# Autodesk Inventor assembly: PCB-HousingAssembly
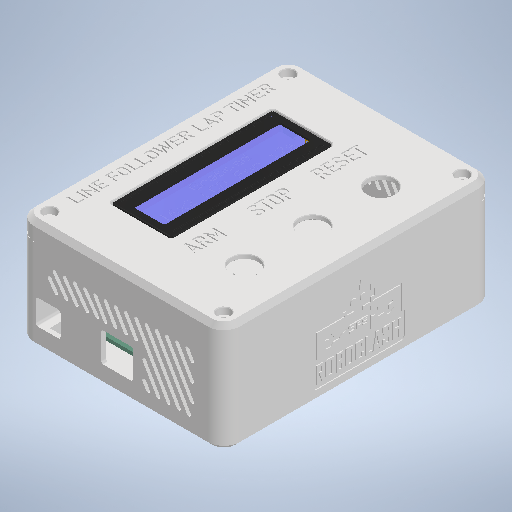
[picture p0: Inventor's stored thumbnail of the model, 512x512]
Saved by Autodesk Inventor 2025.1 (Build 291241000, 241)
## iProperties
Created: 2025-03-29
Part Number: PCB-HousingAssembly
Document SubType Name: Assembly
Designer: 42060
Author: 42060
## Documents named in this file (5)
- C:\Users\42060\Desktop\School\Projects\RoboClash\LineFolloweLapTimer_HousingBottom\PCB-HousingAssembly.iam
- C:\Users\42060\Desktop\School\Projects\RoboClash\LineFolloweLapTimer_HousingBottom\LCD.iam
- C:\Users\42060\Desktop\School\Projects\RoboClash\LineFolloweLapTimer_HousingBottom\PCB-HousingBottom.ipt
- C:\Users\42060\Desktop\School\Projects\RoboClash\LineFolloweLapTimer_HousingBottom\PCB-HousingTop.ipt
- C:\Users\42060\Desktop\School\Projects\RoboClash\LineFolloweLapTimer_HousingBottom\LF_LAP_TIMER.iam
## Components (4 placed, 4 different names)
1. LCD:1 [sub-assembly] — Vložit:2, Vložit:3
2. PCB-HousingBottom:1 — Stejný směr:1, Stejný směr:2, Proti sobě:1, Vložit:4, Úhel:1
3. PCB-HousingTop:1 — Vložit:2, Vložit:3, Stejný směr:1, Stejný směr:2, Proti sobě:1
4. LF_LAP_TIMER:1 [sub-assembly] — Vložit:4, Úhel:1
## Relationships (7: Insert 3, Flush 2, Mate 1, Angle 1)
- Vložit:2 [Insert]: LCD:1 ↔ PCB-HousingTop:1
- Vložit:3 [Insert]: LCD:1 ↔ PCB-HousingTop:1
- Stejný směr:1 [Flush]: PCB-HousingBottom:1 ↔ PCB-HousingTop:1
- Stejný směr:2 [Flush]: PCB-HousingBottom:1 ↔ PCB-HousingTop:1
- Proti sobě:1 [Mate]: PCB-HousingBottom:1 ↔ PCB-HousingTop:1
- Vložit:4 [Insert]: PCB-HousingBottom:1 ↔ LF_LAP_TIMER:1
- Úhel:1 [Angle] (180 deg): PCB-HousingBottom:1 ↔ LF_LAP_TIMER:1
